# Autodesk Inventor assembly: Energy_Pack
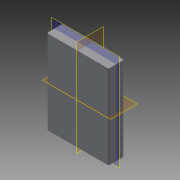
[picture p0: Inventor's stored thumbnail of the model, 180x180]
Saved by Autodesk Inventor 2014 (Build 180170000, 170)
## iProperties
Created: 2015-03-25
Part Number: Energy_Pack
Document SubType Name: Assembly
Designer: Yann
Author: Yann
## Documents named in this file (2)
- C:\Users\Yann\Documents\GitHub\BIKAIR_CAD\Source\Energy_Pack\Energy_Pack.iam
- C:\Users\Yann\Documents\GitHub\BIKAIR_CAD\Source\Energy_Pack\Casing.iam
## Components (1 placed, 1 different names)
1. Casing:1 [sub-assembly] — Affleurement:1, Affleurement:2, Affleurement:3
## Relationships (3: Flush 3)
- Affleurement:1 [Flush]: Casing:1
- Affleurement:2 [Flush]: Casing:1
- Affleurement:3 [Flush]: Casing:1
